# Autodesk Inventor assembly: Montagem4
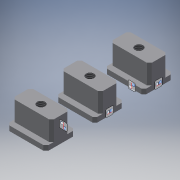
[picture p0: Inventor's stored thumbnail of the model, 180x180]
Saved by Autodesk Inventor 2018 (Build 220112000, 112)
## iProperties
Created: 2018-08-28
Part Number: Montagem4
Material: Genérico
Document SubType Name: Assembly
Designer: Georgines
Author: Georgines
## Documents named in this file (2)
- C:\Users\Georgines\Documents\EstacaoBGA\Peças 3D\Usinagem\Montagem4.iam
- C:\Users\Georgines\Documents\EstacaoBGA\Peças 3D\porcaDeslizante.ipt
## Components (3 placed, 1 different names)
1. porcaDeslizante:1 — Coincidência:1, Alinhamento:10, Alinhamento:11
2. porcaDeslizante:2 — Coincidência:1, Coincidência:2, Alinhamento:9, Alinhamento:10, Alinhamento:11, Alinhamento:12
3. porcaDeslizante:3 — Coincidência:2, Alinhamento:9, Alinhamento:12
## Relationships (6: Flush 4, Mate 2)
- Coincidência:1 [Mate] (8 mm): porcaDeslizante:1 ↔ porcaDeslizante:2
- Coincidência:2 [Mate] (8 mm): porcaDeslizante:2 ↔ porcaDeslizante:3
- Alinhamento:9 [Flush]: porcaDeslizante:2 ↔ porcaDeslizante:3
- Alinhamento:10 [Flush]: porcaDeslizante:1 ↔ porcaDeslizante:2
- Alinhamento:11 [Flush]: porcaDeslizante:1 ↔ porcaDeslizante:2
- Alinhamento:12 [Flush]: porcaDeslizante:2 ↔ porcaDeslizante:3
